# Autodesk Inventor assembly: Slider_crank_mechanism
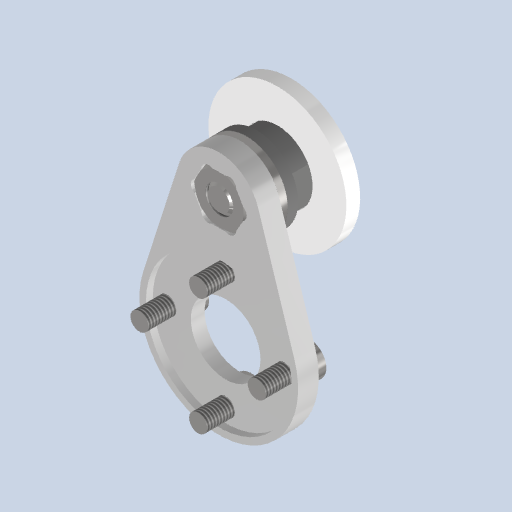
[picture p0: Inventor's stored thumbnail of the model, 512x512]
Saved by Autodesk Inventor 2022 (Build 260153000, 153)
## iProperties
Created: 2022-06-15
Part Number: Slider_crank_mechanism
Document SubType Name: Assembly
Designer: Masato Kubotera
Author: Masato Kubotera
## Documents named in this file (9)
- C:\Users\MasatoKubotera\Desktop\SUSTAINA-OP\LowerBody\Slider_crank\Slider_crank_mechanism.iam
- C:\Users\MasatoKubotera\Desktop\SUSTAINA-OP\LowerBody\Slider_crank\Slider_crank_horn.ipt
- C:\Users\MasatoKubotera\Desktop\SUSTAINA-OP\ReadyMade\InsertNut\S4-05-3W.ipt
- C:\Users\MasatoKubotera\Desktop\SUSTAINA-OP\ReadyMade\Washer\TT-1020-20.ipt
- C:\Users\MasatoKubotera\Desktop\SUSTAINA-OP\ReadyMade\Washer\UUW-0412-10H.ipt
- C:\Users\MasatoKubotera\Desktop\SUSTAINA-OP\ReadyMade\Washer\UUW-0614-05BH.ipt
- C:\Users\MasatoKubotera\Desktop\SUSTAINA-OP\ReadyMade\Bush\LED-0606.ipt
- C:\Users\MasatoKubotera\Desktop\SUSTAINA-OP\ReadyMade\Screw\DBTS4-7-4-DHC.ipt
- C:\Users\MasatoKubotera\Desktop\SUSTAINA-OP\ReadyMade\Screw\LowHead_M2_6-6.ipt
## Components (11 placed, 8 different names)
1. Slider_crank_horn:1 — フラッシュ:1, フラッシュ:2, フラッシュ:3, 挿入:1, 角度:1, 挿入:2, 角度:2, 挿入:7, 挿入:8, 挿入:9, 挿入:10
2. S4-05-3W:1 — 挿入:1, 角度:1
3. TT-1020-20:1 — 挿入:6
4. UUW-0412-10H:1 — 挿入:2, 挿入:3, 挿入:4
5. UUW-0614-05BH:1 — 挿入:5, 挿入:6
6. LED-0606:1 — 挿入:3, 角度:2
7. DBTS4-7-4-DHC:1 — 挿入:4, 挿入:5
8. LowHead_M2_6-6:1 — 挿入:7
9. LowHead_M2_6-6:2 — 挿入:8
10. LowHead_M2_6-6:3 — 挿入:9
11. LowHead_M2_6-6:4 — 挿入:10
## Relationships (15: Insert 10, Flush 3, Angle 2)
- フラッシュ:1 [Flush]: Slider_crank_horn:1
- フラッシュ:2 [Flush]: Slider_crank_horn:1
- フラッシュ:3 [Flush]: Slider_crank_horn:1
- 挿入:1 [Insert]: Slider_crank_horn:1 ↔ S4-05-3W:1
- 角度:1 [Angle] (0 deg): Slider_crank_horn:1 ↔ S4-05-3W:1
- 挿入:2 [Insert]: Slider_crank_horn:1 ↔ UUW-0412-10H:1
- 挿入:3 [Insert]: UUW-0412-10H:1 ↔ LED-0606:1
- 角度:2 [Angle] (0 deg): Slider_crank_horn:1 ↔ LED-0606:1
- 挿入:4 [Insert]: UUW-0412-10H:1 ↔ DBTS4-7-4-DHC:1
- 挿入:5 [Insert]: UUW-0614-05BH:1 ↔ DBTS4-7-4-DHC:1
- 挿入:6 [Insert]: TT-1020-20:1 ↔ UUW-0614-05BH:1
- 挿入:7 [Insert]: Slider_crank_horn:1 ↔ LowHead_M2_6-6:1
- 挿入:8 [Insert]: Slider_crank_horn:1 ↔ LowHead_M2_6-6:2
- 挿入:9 [Insert]: Slider_crank_horn:1 ↔ LowHead_M2_6-6:3
- 挿入:10 [Insert]: Slider_crank_horn:1 ↔ LowHead_M2_6-6:4
